# Autodesk Inventor assembly: Claw assmebly
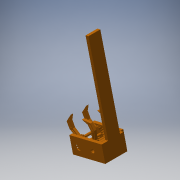
[picture p0: Inventor's stored thumbnail of the model, 180x180]
Saved by Autodesk Inventor 2017 (Build 210142000, 142)
## iProperties
Created: 2018-01-10
Part Number: Claw assmebly
Document SubType Name: Assembly
Designer: Delta
Author: Delta
## Documents named in this file (5)
- C:\Robotics\CAD\2017-18_CAD\Claw assmebly.iam
- C:\Robotics\CAD\2017-18_CAD\Relic arm front.ipt
- C:\Robotics\CAD\2017-18_CAD\Relic Claw.ipt
- C:\Robotics\CAD\2017-18_CAD\servo attachment claw.ipt
- C:\Robotics\CAD\2017-18_CAD\claw attachment back.ipt
## Components (4 placed, 4 different names)
1. servo attachment claw:1 — Mate:2, Mate:3
2. claw attachment back:1 — Mate:4
3. Relic Claw:1 — Mate:2, Mate:3
4. Relic arm front:1 — Mate:4
## Relationships (3: Mate 3)
- Mate:2: servo attachment claw:1 ↔ Relic Claw:1
- Mate:3: servo attachment claw:1 ↔ Relic Claw:1
- Mate:4: claw attachment back:1 ↔ Relic arm front:1
